# Autodesk Inventor assembly: Assembly233
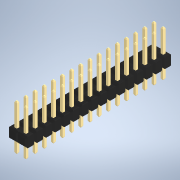
[picture p0: Inventor's stored thumbnail of the model, 180x180]
Saved by Autodesk Inventor 2021 (Build 250183000, 183)
## iProperties
Created: 2023-08-07
Part Number: Assembly233
Document SubType Name: Assembly
Designer: michal
Author: michal
## Documents named in this file (2)
- C:\Users\micha\OneDrive\Dokumenty\GitHub\escape_room_hw_v2\Enclosure\Commercial\Assembly233.iam
- C:\Users\micha\OneDrive\Dokumenty\GitHub\escape_room_hw_v2\Enclosure\Commercial\J10.iam
## Components (32 placed, 1 different names)
1. J10:1 [sub-assembly]
2. J10:2 [sub-assembly]
3. J10:3 [sub-assembly]
4. J10:4 [sub-assembly]
5. J10:5 [sub-assembly]
6. J10:6 [sub-assembly]
7. J10:7 [sub-assembly]
8. J10:8 [sub-assembly]
9. J10:9 [sub-assembly]
10. J10:10 [sub-assembly]
11. J10:11 [sub-assembly]
12. J10:12 [sub-assembly]
13. J10:13 [sub-assembly]
14. J10:14 [sub-assembly]
15. J10:15 [sub-assembly]
16. J10:16 [sub-assembly]
17. J10:17 [sub-assembly]
18. J10:18 [sub-assembly]
19. J10:19 [sub-assembly]
20. J10:20 [sub-assembly]
21. J10:21 [sub-assembly]
22. J10:22 [sub-assembly]
23. J10:23 [sub-assembly]
24. J10:24 [sub-assembly]
25. J10:25 [sub-assembly]
26. J10:26 [sub-assembly]
27. J10:27 [sub-assembly]
28. J10:28 [sub-assembly]
29. J10:29 [sub-assembly]
30. J10:30 [sub-assembly]
31. J10:31 [sub-assembly]
32. J10:32 [sub-assembly]
## Component patterns: (32 elements, first: J10:1)
